# Autodesk Inventor assembly: FINAL Assembly
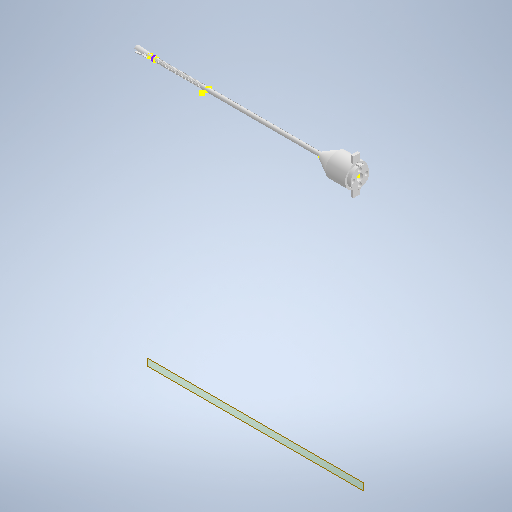
[picture p0: Inventor's stored thumbnail of the model, 512x512]
Saved by Autodesk Inventor 2025.2 (Build 292293000, 293)
## iProperties
Created: 2025-04-03
Part Number: FINAL Assembly
Document SubType Name: Assembly
Designer: avnr2
Author: avnr2
## Documents named in this file (4)
- C:\Users\avnr2\OneDrive\Desktop\CAD- desgin tool\FINAL Assembly.iam
- C:\Users\avnr2\OneDrive\Desktop\CAD- desgin tool\Joy stick part 2.ipt
- C:\Users\avnr2\OneDrive\Desktop\CAD- desgin tool\joy stick part 1.ipt
- C:\Users\avnr2\OneDrive\Desktop\CAD- desgin tool\main tool.ipt
## Components (3 placed, 3 different names)
1. Joy stick part 2:1 — Mate:1
2. joy stick part 1:1
3. main tool:4 — Mate:1
## Relationships (1: Mate 1)
- Mate:1: Joy stick part 2:1 ↔ main tool:4
